# Autodesk Inventor assembly: bellows_2
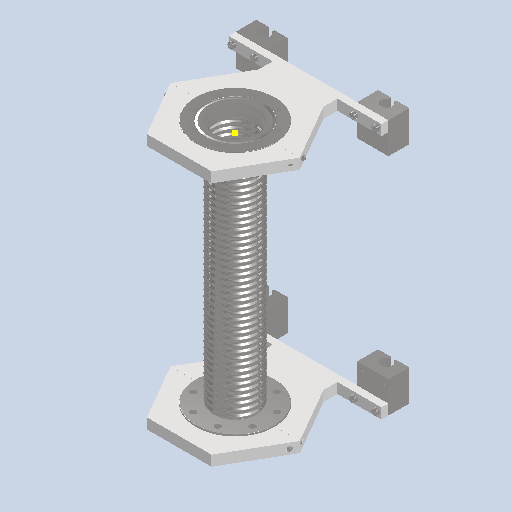
[picture p0: Inventor's stored thumbnail of the model, 512x512]
Saved by Autodesk Inventor 2026.3 (Build 303398000, 398)
## iProperties
Created: 2026-06-24
Part Number: bellows_2
Document SubType Name: Assembly
Designer: shusu
Author: shusu
## Documents named in this file (3)
- C:\Users\shusu\aklab_pihti\PIHTI\bellows\bellows_2.iam
- C:\Users\shusu\aklab_pihti\PIHTI\bellows\bellows_bellows.ipt
- C:\Users\shusu\aklab_pihti\PIHTI\bellows\bellows_1.iam
## Components (3 placed, 2 different names)
1. bellows_bellows:1 — 挿入:1, 挿入:2
2. bellows_1:1 [sub-assembly] — 挿入:2, 角度:1
3. bellows_1:2 [sub-assembly] — 挿入:1, 角度:1
## Relationships (3: Insert 2, Angle 1)
- 挿入:1 [Insert] (-1 mm): bellows_bellows:1 ↔ bellows_1:2
- 挿入:2 [Insert] (1 mm): bellows_bellows:1 ↔ bellows_1:1
- 角度:1 [Angle] (0 deg): bellows_1:1 ↔ bellows_1:2
